# Autodesk Inventor assembly: Assembly
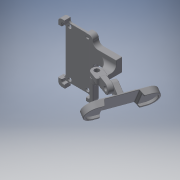
[picture p0: Inventor's stored thumbnail of the model, 180x180]
Saved by Autodesk Inventor 2016 (Build 200138000, 138)
## iProperties
Created: 2019-03-14
Part Number: Assembly
Document SubType Name: Assembly
Designer: HAL-9000
Author: HAL-9000
## Documents named in this file (4)
- C:\Users\HAL-9000\Desktop\Baby and Home Monitoring System\Assembly.iam
- C:\Users\HAL-9000\Desktop\Baby and Home Monitoring System\Wall Mount.ipt
- C:\Users\HAL-9000\Desktop\Baby and Home Monitoring System\Swivel.ipt
- C:\Users\HAL-9000\Desktop\Baby and Home Monitoring System\Camera Mount.ipt
## Components (3 placed, 3 different names)
1. Wall Mount:1 — Insert:1
2. Swivel:1 — Insert:1, Insert:2
3. Camera Mount:1 — Insert:2
## Relationships (2: Insert 2)
- Insert:1: Wall Mount:1 ↔ Swivel:1
- Insert:2: Swivel:1 ↔ Camera Mount:1
